# Autodesk Inventor assembly: Turret Columb Assembly
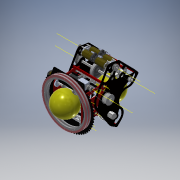
[picture p0: Inventor's stored thumbnail of the model, 180x180]
Saved by Autodesk Inventor 2019.4 (Build 234330000, 330)
## iProperties
Created: 2020-01-18
Part Number: Turret Columb Assembly
Document SubType Name: Assembly
Designer: admin
Mass: 13542.8 g
Surface Area: 20769.1 cm^2
Volume: 12994.1 cm^3
Density: 1.04223 g/cm^3
Author: admin
## Documents named in this file (24)
- C:\Users\Mark\Desktop\7738 Helion Engineering\7738-2020\Robot V2\Turret Columb Assembly\Turret Columb Assembly.iam
- C:\Users\Mark\Desktop\7738 Helion Engineering\7738-2020\Robot V2\Turret\Turret Assembly.iam
- C:\Users\Mark\Desktop\7738 Helion Engineering\7738-2020\Robot V2\Turret Columb Assembly\Column Plate.ipt
- C:\Users\Mark\Desktop\7738 Helion Engineering\7738-2020\Robot V2\Turret Columb Assembly\Slewing Bearing.ipt
- C:\Users\Mark\Desktop\7738 Helion Engineering\7738-2020\Robot V2\Turret Columb Assembly\1001 Gearbox\VersaPlanetary_v1_Two_Stage_100_1_with_BAG.iam
- C:\Users\Mark\Desktop\7738 Helion Engineering\7738-2020\Robot V2\Turret Columb Assembly\Turret Columb Assembly\Design Accelerator\Synchronous Belts Transmission1.iam
- C:\Users\Mark\Desktop\7738 Helion Engineering\7738-2020\Robot V2\Turret Columb Assembly\Turret Columb Assembly\Design Accelerator\Synchronous Belts Transmission2.iam
- C:\Users\Mark\Desktop\7738 Helion Engineering\7738-2020\Robot V2\Turret Columb Assembly\Turret Columb Assembly\Design Accelerator\Synchronous Belts Transmission3.iam
- C:\Users\Mark\Desktop\7738 Helion Engineering\7738-2020\Robot V2\Turret Columb Assembly\Turret Columb Assembly\Design Accelerator\Synchronous Belts Transmission4.iam
- C:\Users\Mark\Desktop\7738 Helion Engineering\7738-2020\Robot V2\Turret Columb Assembly\Bearing Plate.ipt
- C:\Users\Mark\Desktop\7738 Helion Engineering\7738-2020\Robot V2\Turret\F6800.ipt
- C:\Users\Mark\Desktop\7738 Helion Engineering\7738-2020\CAD\F6804zz.ipt
- C:\Users\Mark\Desktop\7738 Helion Engineering\7738-2020\Robot V2\Turret Columb Assembly\Turret Columb Assembly\Design Accelerator\Synchronous Belts Transmission5.iam
- C:\Users\Mark\Desktop\7738 Helion Engineering\7738-2020\Robot V2\Turret\775\775pro_775pro_Connect_and_8T_Pinion_217-6459.iam
- C:\Users\Mark\Desktop\7738 Helion Engineering\7738-2020\Robot V2\Turret\36t_Aluminum_Spur_Gear_20_DP_1_2_Hex_Bore_217-3214.ipt
- C:\Users\Mark\Desktop\7738 Helion Engineering\7738-2020\Robot V2\Turret Columb Assembly\Turret Columb Assembly\Design Accelerator\Synchronous Belts Transmission7.iam
- C:\Users\Mark\Desktop\7738 Helion Engineering\7738-2020\Robot V2\Turret Columb Assembly\Column Axle.ipt
- C:\Users\Mark\Desktop\7738 Helion Engineering\7738-2020\Robot V2\Turret Columb Assembly\Turret Idle Pin.ipt
- C:\Users\Mark\Desktop\7738 Helion Engineering\7738-2020\Robot V2\Turret Columb Assembly\Turret Driven Pin.ipt
- C:\Users\Mark\Desktop\7738 Helion Engineering\7738-2020\Robot V2\Turret Columb Assembly\Bearing Spacer.ipt
- C:\Users\Mark\Desktop\7738 Helion Engineering\7738-2020\Robot V2\Turret Columb Assembly\Column Mount.ipt
- C:\Users\Mark\Desktop\7738 Helion Engineering\7738-2020\Robot V2\Turret Columb Assembly\Column Spacer.ipt
- C:\Users\Mark\Desktop\7738 Helion Engineering\7738-2020\Robot V2\Turret Columb Assembly\Idle Drive Axle.ipt
- C:\Users\Mark\Desktop\7738 Helion Engineering\7738-2020\Power Cell.ipt
## Components (46 placed, 18 different names)
1. Turret Assembly:1 [sub-assembly] — Angle:1, Mate:1, Mate:4, Mate:5, Mate:6, Mate:14, Mate:40, Mate:42
2. Column Plate:1 — Mate:2, Mate:3, Mate:5, Mate:26, Mate:27, Mate:28, Mate:29, Mate:35, Mate:36, Mate:37, Mate:38, Mate:59, Mate:60, Mate:61, Mate:62, Flush:2, Mate:76, Flush:4, Mate:78, Mate:79, Mate:80, Mate:81, Mate:86, Mate:89
3. Column Plate:2 — Mate:2, Mate:3, Mate:4, Mate:6, Angle:2, Mate:17, Mate:20, Mate:21, Mate:23, Mate:24, Mate:25, Mate:30, Mate:31, Mate:32, Mate:33, Mate:34, Mate:41, Mate:43, Mate:45, Mate:75, Flush:3, Mate:82, Mate:83, Mate:84, Mate:85, Mate:87, Mate:88
4. VersaPlanetary_v1_Two_Stage_100_1_with_BAG:1 [sub-assembly] — Angle:3, Mate:44, Flush:2
5. Synchronous Belts Transmission:1 [sub-assembly]
6. Synchronous Belts Transmission:2 [sub-assembly]
7. Synchronous Belts Transmission:3 [sub-assembly]
8. Slewing Bearing:4 — Mate:14, Angle:2, Mate:15, Mate:16, Mate:17, Mate:19, Mate:39, Mate:64, Mate:65, Mate:66, Mate:67, Mate:93
9. Slewing Bearing:5 — Mate:15, Mate:16, Mate:39, Mate:68, Mate:69, Mate:70, Mate:71, Mate:72
10. Synchronous Belts Transmission:4 [sub-assembly] — Mate:46, Mate:48
11. Bearing Plate:1 — Mate:19, Mate:20, Mate:21, Flush:1, Angle:3, Mate:74, Mate:77
12. F6800:1 — Mate:23, Mate:34
13. F6800:2 — Mate:25, Mate:31, Mate:47, Mate:49, Mate:50
14. F6800:3 — Mate:24, Mate:33
15. F6800:4 — Mate:26, Mate:36
16. F6800:5 — Mate:29, Mate:37
17. F6800:6 — Mate:27, Mate:35, Mate:52, Mate:54
18. F6800:7 — Mate:30, Mate:32, Mate:51, Mate:56
19. F6800:8 — Mate:28, Mate:38, Mate:53, Mate:55
20. F6804zz:1 — Mate:41, Mate:43, Mate:58
21. F6804zz:3 — Mate:40, Mate:42, Mate:57
22. Synchronous Belts Transmission:5 [sub-assembly] — Mate:44
23. 775pro_775pro_Connect_and_8T_Pinion_217-6459:1 [sub-assembly] — Mate:45, Mate:48
24. 36t_Aluminum_Spur_Gear_20_DP_1_2_Hex_Bore_217-3214:1 — Mate:46, Mate:47
25. Synchronous Belts Transmission:6 [sub-assembly]
26. Column Axle:1 — Mate:53, Mate:55
27. Column Axle:2 — Mate:52, Mate:54
28. Column Axle:3 — Mate:51, Mate:56
29. Column Axle:4 — Mate:49, Mate:50
30. Turret Idle Pin:1 — Mate:57, Mate:58
31. Turret Driven Pin:1 — Mate:59, Mate:60, Mate:63
32. F6804zz:4 — Mate:61, Mate:62, Mate:63
33. Bearing Spacer:1 — Mate:70, Mate:71, Mate:72, Mate:73
34. Bearing Spacer:2 — Mate:68, Mate:69
35. Bearing Spacer:3 — Mate:66, Mate:67, Mate:73
36. Bearing Spacer:4 — Mate:64, Mate:65
37. Column Mount:1 — Mate:74, Mate:75, Flush:3
38. Column Mount:2 — Mate:76, Mate:77, Flush:4
39. Column Spacer:1 — Mate:78, Mate:84
40. Column Spacer:2 — Mate:79, Mate:85
41. Column Spacer:3 — Mate:80, Mate:83
42. Column Spacer:4 — Mate:81, Mate:82
43. F6800:9 — Mate:86, Mate:89, Mate:90, Mate:91
44. F6800:10 — Mate:87, Mate:88
45. Idle Drive Axle:1 — Mate:90, Mate:91
46. Power Cell:1 — Mate:92, Mate:93
## Relationships (91: Mate 84, Flush 4, Angle 3)
- Angle:1 (65 deg): Turret Assembly:1
- Mate:1: Turret Assembly:1
- Mate:2: Column Plate:1 ↔ Column Plate:2
- Mate:3: Column Plate:1 ↔ Column Plate:2
- Mate:4 (5 mm): Turret Assembly:1 ↔ Column Plate:2
- Mate:5 (5 mm): Turret Assembly:1 ↔ Column Plate:1
- Mate:6: Turret Assembly:1 ↔ Column Plate:2
- Mate:14: Turret Assembly:1 ↔ Slewing Bearing:4
- Angle:2 (0 deg): Column Plate:2 ↔ Slewing Bearing:4
- Mate:15: Slewing Bearing:4 ↔ Slewing Bearing:5
- Mate:16 (11.6 mm): Slewing Bearing:4 ↔ Slewing Bearing:5
- Mate:17 (173 mm): Column Plate:2 ↔ Slewing Bearing:4
- Mate:19 (3 mm): Slewing Bearing:4 ↔ Bearing Plate:1
- Mate:20 (1 mm): Column Plate:2 ↔ Bearing Plate:1
- Mate:21 (1 mm): Column Plate:2 ↔ Bearing Plate:1
- Flush:1 (21 mm): Bearing Plate:1
- Mate:23: Column Plate:2 ↔ F6800:1
- Mate:24: Column Plate:2 ↔ F6800:3
- Mate:25: Column Plate:2 ↔ F6800:2
- Mate:26: Column Plate:1 ↔ F6800:4
- Mate:27: Column Plate:1 ↔ F6800:6
- Mate:28: Column Plate:1 ↔ F6800:8
- Mate:29: Column Plate:1 ↔ F6800:5
- Mate:30: Column Plate:2 ↔ F6800:7
- Mate:31 (0.2 mm): Column Plate:2 ↔ F6800:2
- Mate:32 (0.2 mm): Column Plate:2 ↔ F6800:7
- Mate:33 (0.2 mm): Column Plate:2 ↔ F6800:3
- Mate:34 (0.2 mm): Column Plate:2 ↔ F6800:1
- Mate:35 (0.2 mm): Column Plate:1 ↔ F6800:6
- Mate:36 (0.2 mm): Column Plate:1 ↔ F6800:4
- Mate:37 (0.2 mm): Column Plate:1 ↔ F6800:5
- Mate:38 (0.2 mm): Column Plate:1 ↔ F6800:8
- Angle:3 (0 deg): VersaPlanetary_v1_Two_Stage_100_1_with_BAG:1 ↔ Bearing Plate:1
- Mate:39: Slewing Bearing:4 ↔ Slewing Bearing:5
- Mate:40: Turret Assembly:1 ↔ F6804zz:3
- Mate:41: Column Plate:2 ↔ F6804zz:1
- Mate:42 (0.2 mm): Turret Assembly:1 ↔ F6804zz:3
- Mate:43 (0.2 mm): Column Plate:2 ↔ F6804zz:1
- Mate:44: VersaPlanetary_v1_Two_Stage_100_1_with_BAG:1 ↔ Synchronous Belts Transmission:5
- Mate:45: Column Plate:2 ↔ 775pro_775pro_Connect_and_8T_Pinion_217-6459:1
- Mate:46: Synchronous Belts Transmission:4 ↔ 36t_Aluminum_Spur_Gear_20_DP_1_2_Hex_Bore_217-3214:1
- Mate:47 (2 mm): F6800:2 ↔ 36t_Aluminum_Spur_Gear_20_DP_1_2_Hex_Bore_217-3214:1
- Mate:48 (29.21 mm): Synchronous Belts Transmission:4 ↔ 775pro_775pro_Connect_and_8T_Pinion_217-6459:1
- Mate:49: F6800:2 ↔ Column Axle:4
- Mate:50 (0.1 mm): F6800:2 ↔ Column Axle:4
- Mate:51: F6800:7 ↔ Column Axle:3
- Mate:52: F6800:6 ↔ Column Axle:2
- Mate:53: F6800:8 ↔ Column Axle:1
- Mate:54 (0.1 mm): F6800:6 ↔ Column Axle:2
- Mate:55 (0.1 mm): F6800:8 ↔ Column Axle:1
- Mate:56 (0.1 mm): F6800:7 ↔ Column Axle:3
- Mate:57: F6804zz:3 ↔ Turret Idle Pin:1
- Mate:58: F6804zz:1 ↔ Turret Idle Pin:1
- Mate:59: Column Plate:1 ↔ Turret Driven Pin:1
- Mate:60: Column Plate:1 ↔ Turret Driven Pin:1
- Mate:61: Column Plate:1 ↔ F6804zz:4
- Mate:62 (0.2 mm): Column Plate:1 ↔ F6804zz:4
- Mate:63: Turret Driven Pin:1 ↔ F6804zz:4
- Mate:64: Slewing Bearing:4 ↔ Bearing Spacer:4
- Mate:65: Slewing Bearing:4 ↔ Bearing Spacer:4
- Mate:66: Slewing Bearing:4 ↔ Bearing Spacer:3
- Mate:67: Slewing Bearing:4 ↔ Bearing Spacer:3
- Mate:68: Slewing Bearing:5 ↔ Bearing Spacer:2
- Mate:69: Slewing Bearing:5 ↔ Bearing Spacer:2
- Mate:70: Slewing Bearing:5 ↔ Bearing Spacer:1
- Mate:71: Slewing Bearing:5 ↔ Bearing Spacer:1
- Mate:72: Slewing Bearing:5 ↔ Bearing Spacer:1
- Mate:73: Bearing Spacer:1 ↔ Bearing Spacer:3
- Flush:2 (-6 mm): Column Plate:1 ↔ VersaPlanetary_v1_Two_Stage_100_1_with_BAG:1
- Mate:74: Bearing Plate:1 ↔ Column Mount:1
- Mate:75: Column Plate:2 ↔ Column Mount:1
- Flush:3 (30 mm): Column Plate:2 ↔ Column Mount:1
- Mate:76: Column Plate:1 ↔ Column Mount:2
- Mate:77: Bearing Plate:1 ↔ Column Mount:2
- Flush:4 (30 mm): Column Plate:1 ↔ Column Mount:2
- Mate:78: Column Plate:1 ↔ Column Spacer:1
- Mate:79: Column Plate:1 ↔ Column Spacer:2
- Mate:80: Column Plate:1 ↔ Column Spacer:3
- Mate:81: Column Plate:1 ↔ Column Spacer:4
- Mate:82: Column Plate:2 ↔ Column Spacer:4
- Mate:83: Column Plate:2 ↔ Column Spacer:3
- Mate:84: Column Plate:2 ↔ Column Spacer:1
- Mate:85: Column Plate:2 ↔ Column Spacer:2
- Mate:86: Column Plate:1 ↔ F6800:9
- Mate:87: Column Plate:2 ↔ F6800:10
- Mate:88 (0.2 mm): Column Plate:2 ↔ F6800:10
- Mate:89 (0.2 mm): Column Plate:1 ↔ F6800:9
- Mate:90: F6800:9 ↔ Idle Drive Axle:1
- Mate:91: F6800:9 ↔ Idle Drive Axle:1
- Mate:92: Power Cell:1
- Mate:93: Slewing Bearing:4 ↔ Power Cell:1
